# Autodesk Inventor assembly: Shoulder
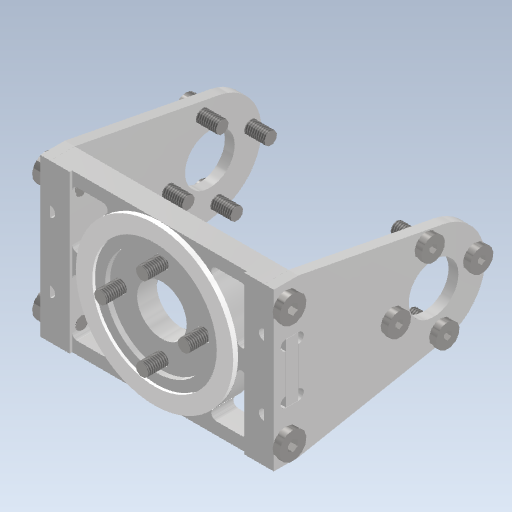
[picture p0: Inventor's stored thumbnail of the model, 512x512]
Saved by Autodesk Inventor 2020 (Build 240168000, 168)
## iProperties
Created: 2021-09-24
Part Number: Shoulder
Document SubType Name: Assembly
Designer: Masato Kubotera
Mass: 26.1068 g
Surface Area: 95.2903 cm^2
Volume: 8.79774 cm^3
Density: 2.96744 g/cm^3
Author: Masato Kubotera
## Documents named in this file (7)
- C:\Users\Masato\Documents\Inventor\CIT Brains_Inventor\OpenPlatform_ver3_0 - Ver4_1branch\UpperBody\Arm\Shoulder.iam
- C:\Users\Masato\Documents\Inventor\CIT Brains_Inventor\OpenPlatform_ver3_0 - Ver4_1branch\UpperBody\Arm\Shoulder_horn_frame.ipt
- C:\Users\Masato\Documents\Inventor\CIT Brains_Inventor\OpenPlatform_ver3_0 - Ver4_1branch\UpperBody\Arm\Shoulder_side_frame.ipt
- C:\Users\Masato\Documents\Inventor\CIT Brains_Inventor\OpenPlatform_ver3_0 - Ver4_1branch\Ready_Made\Screw\M3-6.ipt
- C:\Users\Masato\Documents\Inventor\CIT Brains_Inventor\OpenPlatform_ver3_0\Ready_Made\TT-2532-10.ipt
- C:\Users\Masato\Documents\Inventor\CIT Brains_Inventor\OpenPlatform_ver3_0 - Ver4_1branch\Ready_Made\Screw\M2_6-6.ipt
- C:\Users\Masato\Documents\Inventor\CIT Brains_Inventor\OpenPlatform_ver3_0 - Ver4_1branch\Ready_Made\Screw\M2_6-8.ipt
## Components (20 placed, 6 different names)
1. Shoulder_horn_frame:1 — 挿入:1, 挿入:2, 挿入:9, 挿入:10, 挿入:11, 挿入:22, 挿入:23, 挿入:24, 挿入:25
2. Shoulder_side_frame:1 — 挿入:1, 挿入:2, 挿入:7, 挿入:8, 挿入:18, 挿入:19, 挿入:20, 挿入:21
3. Shoulder_side_frame:2 — 挿入:10, 挿入:11, 挿入:12, 挿入:13, 挿入:14, 挿入:15, 挿入:16, 挿入:17
4. M3-6:1 — 挿入:12
5. M3-6:2 — 挿入:13
6. M3-6:3 — 挿入:7
7. M3-6:4 — 挿入:8
8. TT-2532-10:1 — 挿入:9
9. M2_6-6:1 — 挿入:14
10. M2_6-6:2 — 挿入:15
11. M2_6-6:3 — 挿入:16
12. M2_6-6:4 — 挿入:17
13. M2_6-6:5 — 挿入:18
14. M2_6-6:6 — 挿入:19
15. M2_6-6:7 — 挿入:20
16. M2_6-6:8 — 挿入:21
17. M2_6-8:1 — 挿入:22
18. M2_6-8:2 — 挿入:23
19. M2_6-8:3 — 挿入:24
20. M2_6-8:4 — 挿入:25
## Relationships (21: Insert 21)
- 挿入:1 [Insert]: Shoulder_horn_frame:1 ↔ Shoulder_side_frame:1
- 挿入:2 [Insert]: Shoulder_horn_frame:1 ↔ Shoulder_side_frame:1
- 挿入:7 [Insert]: Shoulder_side_frame:1 ↔ M3-6:3
- 挿入:8 [Insert]: Shoulder_side_frame:1 ↔ M3-6:4
- 挿入:9 [Insert]: Shoulder_horn_frame:1 ↔ TT-2532-10:1
- 挿入:10 [Insert]: Shoulder_horn_frame:1 ↔ Shoulder_side_frame:2
- 挿入:11 [Insert]: Shoulder_horn_frame:1 ↔ Shoulder_side_frame:2
- 挿入:12 [Insert]: Shoulder_side_frame:2 ↔ M3-6:1
- 挿入:13 [Insert]: Shoulder_side_frame:2 ↔ M3-6:2
- 挿入:14 [Insert]: Shoulder_side_frame:2 ↔ M2_6-6:1
- 挿入:15 [Insert]: Shoulder_side_frame:2 ↔ M2_6-6:2
- 挿入:16 [Insert]: Shoulder_side_frame:2 ↔ M2_6-6:3
- 挿入:17 [Insert]: Shoulder_side_frame:2 ↔ M2_6-6:4
- 挿入:18 [Insert]: Shoulder_side_frame:1 ↔ M2_6-6:5
- 挿入:19 [Insert]: Shoulder_side_frame:1 ↔ M2_6-6:6
- 挿入:20 [Insert]: Shoulder_side_frame:1 ↔ M2_6-6:7
- 挿入:21 [Insert]: Shoulder_side_frame:1 ↔ M2_6-6:8
- 挿入:22 [Insert]: Shoulder_horn_frame:1 ↔ M2_6-8:1
- 挿入:23 [Insert]: Shoulder_horn_frame:1 ↔ M2_6-8:2
- 挿入:24 [Insert]: Shoulder_horn_frame:1 ↔ M2_6-8:3
- 挿入:25 [Insert]: Shoulder_horn_frame:1 ↔ M2_6-8:4
